# Autodesk Inventor assembly: Assembly
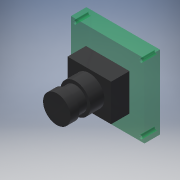
[picture p0: Inventor's stored thumbnail of the model, 180x180]
Saved by Autodesk Inventor 2016 (Build 200138000, 138)
## iProperties
Created: 2016-04-14
Part Number: Assembly
Document SubType Name: Assembly
Designer: Andres
Author: Andres
## Documents named in this file (3)
- \\Mac\Home\Documents\repositorios\BoreholeCamera\CAD_Probe\Camera\Assembly\Assembly.iam
- Z:\Documents\repositorios\BoreholeCamera\CAD_Probe\Camera\PCB_Camera.ipt
- Z:\Documents\repositorios\BoreholeCamera\CAD_Probe\Camera\Camera.ipt
## Components (2 placed, 2 different names)
1. PCB_Camera:1 — Rigid:1
2. Camera:1 — Rigid:1
## Relationships (1: WeldJoint 1)
- Rigid:1 [WeldJoint]: PCB_Camera:1 ↔ Camera:1
